# Autodesk Inventor assembly: Shoulder
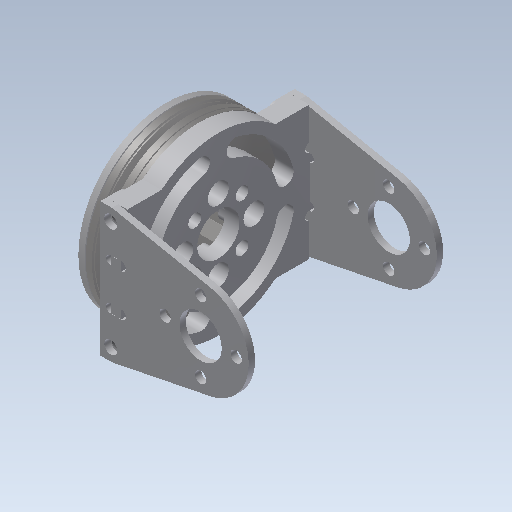
[picture p0: Inventor's stored thumbnail of the model, 512x512]
Saved by Autodesk Inventor 2020.4 (Build 244396000, 396)
## iProperties
Created: 2016-05-05
Part Number: Shoulder
Document SubType Name: Assembly
Designer: hiroaki
Mass: 31.2319 g
Surface Area: 187.261 cm^2
Volume: 14.2636 cm^3
Density: 2.18962 g/cm^3
Author: hiroaki
## Documents named in this file (7)
- C:\Users\Masato\Documents\Inventor\CIT Brains_Inventor\OpenPlatform_ver3_0\UpperBody\Arm\Shoulder.iam
- C:\Users\Masato\Documents\Inventor\CIT Brains_Inventor\OpenPlatform_ver3_0\UpperBody\Arm\Shoulder_vertical_frame_01.ipt
- C:\Users\Masato\Documents\Inventor\CIT Brains_Inventor\OpenPlatform_ver3_0\UpperBody\Arm\Shoulder_vertical_frame_02.ipt
- C:\Users\Masato\Documents\Inventor\CIT Brains_Inventor\OpenPlatform_ver3_0\Ready_Made\BA2542\BA2542.ipt
- C:\Users\Masato\Documents\Inventor\CIT Brains_Inventor\OpenPlatform_ver3_0\Ready_Made\BA2542\BA2542_Washer.ipt
- C:\Users\Masato\Documents\Inventor\CIT Brains_Inventor\OpenPlatform_ver3_0\Ready_Made\MSU-306-03.ipt
- C:\Users\Masato\Documents\Inventor\CIT Brains_Inventor\OpenPlatform_ver3_0\Thrust\Thrust_frame_01.ipt
## Components (11 placed, 6 different names)
1. Shoulder_vertical_frame_01:1 — 挿入:1, 挿入:2, 挿入:3, 挿入:4, 挿入:9, 挿入:16, 挿入:17, 挿入:18, 挿入:19
2. Shoulder_vertical_frame_02:1 — 挿入:3, 挿入:4
3. Shoulder_vertical_frame_02:2 — 挿入:1, 挿入:2
4. core_BA2542:1 — 挿入:10
5. washer_BA2542:1 — 挿入:9, 挿入:10
6. core_BA2542:2 — 挿入:20
7. MSU-306-03:1 — 挿入:16, 挿入:23
8. MSU-306-03:2 — 挿入:17, 挿入:24
9. MSU-306-03:3 — 挿入:18, 挿入:21
10. MSU-306-03:4 — 挿入:19, 挿入:22
11. Thrust_frame_01:1 — 挿入:20, 挿入:21, 挿入:22, 挿入:23, 挿入:24
## Relationships (15: Insert 15)
- 挿入:1 [Insert]: Shoulder_vertical_frame_01:1 ↔ Shoulder_vertical_frame_02:2
- 挿入:2 [Insert]: Shoulder_vertical_frame_01:1 ↔ Shoulder_vertical_frame_02:2
- 挿入:3 [Insert]: Shoulder_vertical_frame_01:1 ↔ Shoulder_vertical_frame_02:1
- 挿入:4 [Insert]: Shoulder_vertical_frame_01:1 ↔ Shoulder_vertical_frame_02:1
- 挿入:9 [Insert]: Shoulder_vertical_frame_01:1 ↔ washer_BA2542:1
- 挿入:10 [Insert]: core_BA2542:1 ↔ washer_BA2542:1
- 挿入:16 [Insert]: Shoulder_vertical_frame_01:1 ↔ MSU-306-03:1
- 挿入:17 [Insert]: Shoulder_vertical_frame_01:1 ↔ MSU-306-03:2
- 挿入:18 [Insert]: Shoulder_vertical_frame_01:1 ↔ MSU-306-03:3
- 挿入:19 [Insert]: Shoulder_vertical_frame_01:1 ↔ MSU-306-03:4
- 挿入:20 [Insert]: core_BA2542:2 ↔ Thrust_frame_01:1
- 挿入:21 [Insert]: MSU-306-03:3 ↔ Thrust_frame_01:1
- 挿入:22 [Insert]: MSU-306-03:4 ↔ Thrust_frame_01:1
- 挿入:23 [Insert]: MSU-306-03:1 ↔ Thrust_frame_01:1
- 挿入:24 [Insert]: MSU-306-03:2 ↔ Thrust_frame_01:1
